# Autodesk Inventor assembly: speed_measuring_V1
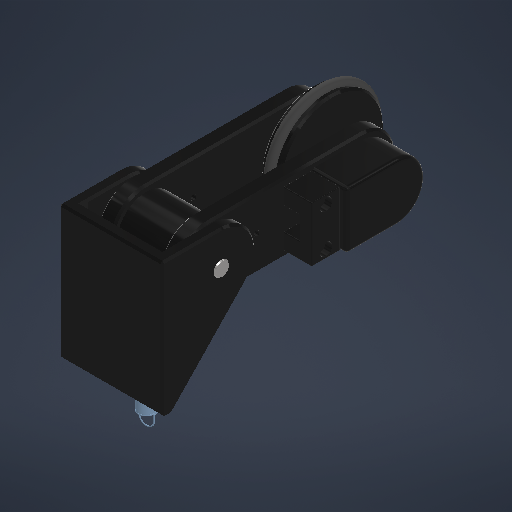
[picture p0: Inventor's stored thumbnail of the model, 512x512]
Saved by Autodesk Inventor 2026 (Build 300175000, 175)
## iProperties
Created: 2023-02-13
Part Number: speed_measuring_V1
Document SubType Name: Assembly
Designer: Mathi
Author: Mathi
## Documents named in this file (13)
- C:\Users\Mathi\sciebo\04_Research\03_Completed projects\2022_03_Tiptop\03_Bicycle-Simulator\02_Simulator_Design\CAD designs\speed\speed_measuring_V1.iam
- C:\Users\Mathi\sciebo\06_Personal\Mathis_Linnenbrink\CAD_archive\Bicycle Simulator\speed_wheel\DIN-988_d8_D14_t02.ipt
- C:\Users\Mathi\sciebo\04_Research\03_Completed projects\2022_03_Tiptop\03_Bicycle-Simulator\02_Simulator_Design\CAD designs\speed\measuring_wheel_V1.ipt
- C:\Users\Mathi\sciebo\04_Research\03_Completed projects\2022_03_Tiptop\03_Bicycle-Simulator\02_Simulator_Design\CAD designs\speed\HEDM-5500_13_V1.ipt
- C:\Users\Mathi\sciebo\04_Research\03_Completed projects\2022_03_Tiptop\03_Bicycle-Simulator\02_Simulator_Design\CAD designs\speed\sealing_ring_V1.ipt
- C:\Users\Mathi\sciebo\04_Research\03_Completed projects\2022_03_Tiptop\03_Bicycle-Simulator\02_Simulator_Design\CAD designs\speed\F688ZZ_V1.ipt
- C:\Users\Mathi\sciebo\04_Research\03_Completed projects\2022_03_Tiptop\03_Bicycle-Simulator\02_Simulator_Design\CAD designs\speed\DIN-988_d8_D14_t02_V1.ipt
- C:\Users\Mathi\sciebo\04_Research\03_Completed projects\2022_03_Tiptop\03_Bicycle-Simulator\02_Simulator_Design\CAD designs\speed\pos-ring_d8_D12_t5_M3_V1.ipt
- C:\Users\Mathi\sciebo\04_Research\03_Completed projects\2022_03_Tiptop\03_Bicycle-Simulator\02_Simulator_Design\CAD designs\speed\wheel_shaft_D8_V1.ipt
- C:\Users\Mathi\sciebo\04_Research\03_Completed projects\2022_03_Tiptop\03_Bicycle-Simulator\02_Simulator_Design\CAD designs\speed\lever_V1.ipt
- C:\Users\Mathi\sciebo\04_Research\03_Completed projects\2022_03_Tiptop\03_Bicycle-Simulator\02_Simulator_Design\CAD designs\speed\joint_flange_V1.ipt
- C:\Users\Mathi\sciebo\04_Research\03_Completed projects\2022_03_Tiptop\03_Bicycle-Simulator\02_Simulator_Design\CAD designs\speed\connector_securing_V1.ipt
- C:\Users\Mathi\sciebo\04_Research\03_Completed projects\2022_03_Tiptop\03_Bicycle-Simulator\02_Simulator_Design\CAD designs\speed\RZ-054AI.ipt
## Components (20 placed, 12 different names)
1. measuring_wheel_V1:1 — Passend:1, Passend:2, Passend:12, Passend:15
2. HEDM-5500_13_V1:1 — Passend:5, Passend:21, Passend:22, Passend:28, Passend:29
3. sealing_ring_V1:1 — Passend:3, Passend:4
4. F688ZZ_V1:1 — Passend:7, Passend:10
5. F688ZZ_V1:2
6. DIN-988_d8_D14_t02_V1:1 — Passend:8, Passend:10, Passend:12
7. pos-ring_d8_D12_t5_M3_V1:1 — Passend:13, Passend:14, Passend:15, Passend:16
8. wheel_shaft_D8_V1:1 — Passend:17, Passend:18
9. lever_V1:1 — Passend:19, Passend:20, Passend:21, Passend:22, Passend:24, Passend:27
10. joint_flange_V1:1 — Passend:24, Passend:25, Passend:26, Insert:1
11. connector_securing_V1:1 — Passend:27, Passend:28, Passend:29
12. wheel_shaft_D8_V1:2 — Insert:1
13. RZ-054AI:1
14. DIN-988_d8_D14_t02:1 — Passend:8, Passend:9, Passend:16
15. DIN-988_d8_D14_t02:3
16. DIN-988_d8_D14_t02:4
17. DIN-988_d8_D14_t02:5
18. DIN-988_d8_D14_t02:6
19. DIN-988_d8_D14_t02:7
20. DIN-988_d8_D14_t02:8
## Component patterns: (7 elements, first: DIN-988_d8_D14_t02:1)
## Relationships (29: Mate 28, Insert 1)
- Passend:1 [Mate]: measuring_wheel_V1:1
- Passend:2 [Mate]: measuring_wheel_V1:1
- Passend:3 [Mate]: sealing_ring_V1:1
- Passend:4 [Mate]: sealing_ring_V1:1
- Passend:5 [Mate]: HEDM-5500_13_V1:1
- [Mate]: F688ZZ_V1:1 ↔ F688ZZ_V1:2
- Passend:7 [Mate]: F688ZZ_V1:1
- Passend:8 [Mate]: DIN-988_d8_D14_t02_V1:1 ↔ DIN-988_d8_D14_t02:1
- Passend:9 [Mate]: DIN-988_d8_D14_t02:1
- Passend:10 [Mate]: F688ZZ_V1:1 ↔ DIN-988_d8_D14_t02_V1:1
- Passend:12 [Mate]: measuring_wheel_V1:1 ↔ DIN-988_d8_D14_t02_V1:1
- Passend:13 [Mate]: pos-ring_d8_D12_t5_M3_V1:1
- Passend:14 [Mate]: pos-ring_d8_D12_t5_M3_V1:1
- Passend:15 [Mate]: measuring_wheel_V1:1 ↔ pos-ring_d8_D12_t5_M3_V1:1
- Passend:16 [Mate]: pos-ring_d8_D12_t5_M3_V1:1 ↔ DIN-988_d8_D14_t02:1
- Passend:17 [Mate]: wheel_shaft_D8_V1:1
- Passend:18 [Mate]: wheel_shaft_D8_V1:1
- Passend:19 [Mate]: lever_V1:1
- Passend:20 [Mate]: lever_V1:1
- Passend:21 [Mate]: HEDM-5500_13_V1:1 ↔ lever_V1:1
- Passend:22 [Mate]: HEDM-5500_13_V1:1 ↔ lever_V1:1
- [Mate]: F688ZZ_V1:2 ↔ lever_V1:1
- Passend:24 [Mate]: lever_V1:1 ↔ joint_flange_V1:1
- Passend:25 [Mate]: joint_flange_V1:1
- Passend:26 [Mate]: joint_flange_V1:1
- Passend:27 [Mate]: lever_V1:1 ↔ connector_securing_V1:1
- Passend:28 [Mate]: HEDM-5500_13_V1:1 ↔ connector_securing_V1:1
- Passend:29 [Mate]: HEDM-5500_13_V1:1 ↔ connector_securing_V1:1
- Insert:1: joint_flange_V1:1 ↔ wheel_shaft_D8_V1:2
